# Autodesk Inventor assembly: Bend Piece 1764
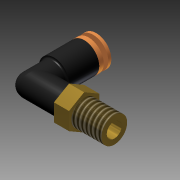
[picture p0: Inventor's stored thumbnail of the model, 180x180]
Saved by Autodesk Inventor 2011 (Build 150239000, 239)
## iProperties
Created: 2010-02-15
Part Number: Bend Piece 1764
Document SubType Name: Assembly
Designer: jgehrig
Author: jgehrig
## Documents named in this file (4)
- R:\CAD Archives\Pnewmatics\Seloniod 1764\Pnewmatics Bend Piece 1764\Pnewmatic Bend Piece 1764.iam
- R:\CAD Archives\Pnewmatics\Seloniod 1764\Pnewmatics Bend Piece 1764\Pnematic Screw Part 1764.ipt
- R:\CAD Archives\Pnewmatics\Seloniod 1764\Pnewmatics Bend Piece 1764\Pnewmatic Screw Part 2 1764.ipt
- R:\CAD Archives\Pnewmatics\Pnewmatics Bend Piece 1764\Pnewmatic Bend Piece 1764.ipt
## Components (3 placed, 3 different names)
1. Pnewmatic Bend Piece 1764:1 — Insert:1, Insert:2
2. Pnematic Screw Part 1764:1 — Insert:2
3. Pnewmatic Screw Part 2 1764:1 — Insert:1
## Relationships (2: Insert 2)
- Insert:1: Pnewmatic Bend Piece 1764:1 ↔ Pnewmatic Screw Part 2 1764:1
- Insert:2: Pnewmatic Bend Piece 1764:1 ↔ Pnematic Screw Part 1764:1
